# Autodesk Inventor assembly: 長穴減速_ホーン
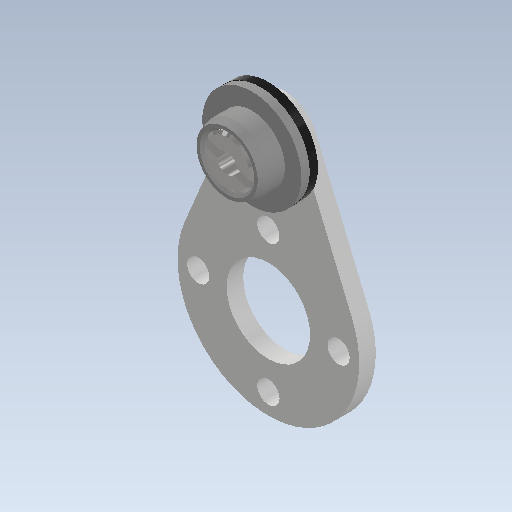
[picture p0: Inventor's stored thumbnail of the model, 512x512]
Saved by Autodesk Inventor 2020 (Build 240168000, 168)
## iProperties
Created: 2021-09-06
Part Number: 長穴減速_ホーン
Document SubType Name: Assembly
Designer: Masato
Mass: 2.53036 g
Surface Area: 18.5815 cm^2
Volume: 1.13409 cm^3
Density: 2.23118 g/cm^3
Author: Masato
## Documents named in this file (5)
- C:\Users\Masato\Desktop\最新版\OpenPlatform_ver3_0\下半身\長穴減速\長穴減速_ホーン.iam
- C:\Users\Masato\Desktop\最新版\OpenPlatform_ver3_0\下半身\長穴減速\長穴減速_ホーン_1.ipt
- C:\Users\Masato\Desktop\最新版\OpenPlatform_ver3_0\Ready_Made\80F-0603.ipt
- C:\Users\Masato\Desktop\最新版\OpenPlatform_ver3_0\Ready_Made\ARU-304S.ipt
- C:\Users\Masato\Desktop\最新版\OpenPlatform_ver3_0\Ready_Made\UUW-0312-10BH.ipt
## Components (4 placed, 4 different names)
1. 長穴減速_ホーン_1:1 — 挿入:1
2. 80F-0603:1 — 挿入:2
3. ARU-304S:1 — 挿入:3
4. UUW-0312-10BH:1 — 挿入:1, 挿入:2, 挿入:3
## Relationships (3: Insert 3)
- 挿入:1 [Insert]: 長穴減速_ホーン_1:1 ↔ UUW-0312-10BH:1
- 挿入:2 [Insert]: 80F-0603:1 ↔ UUW-0312-10BH:1
- 挿入:3 [Insert]: ARU-304S:1 ↔ UUW-0312-10BH:1
